# Autodesk Inventor assembly: 8 Omni Wheel
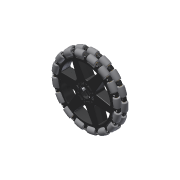
[picture p0: Inventor's stored thumbnail of the model, 180x180]
Saved by Autodesk Inventor 2013 (Build 170138000, 138)
## iProperties
Created: 2013-01-03
Part Number: 8 Omni Wheel
Document SubType Name: Assembly
Designer: Nemo
Author: Nemo
## Documents named in this file (6)
- H:\Nemo\Documents\Robotics\VexPro\Omni Wheel\8 Omni Wheel.iam
- H:\Nemo\Documents\Robotics\VexPro\Omni Wheel\Components\Omni Wheel Inside 8 in.ipt
- H:\Nemo\Documents\Robotics\VexPro\Omni Wheel\Components\Omni Wheel Outside 8 in.ipt
- H:\Nemo\Documents\Robotics\VexPro\Fasteners\Hex Standoff 8-32 x750.ipt
- H:\Nemo\Documents\Robotics\VexPro\Wheels\Components\Omni Roller 8 in.iam
- H:\Nemo\Documents\Robotics\VexPro\Omni Wheel\Components\Omni Wheel Screw for VexPro.ipt
## Components (73 placed, 5 different names)
1. Omni Wheel Inside 8 in:1 — Mate:1, Mate:3, Mate:4, Mate:5, Mate:7, Mate:8, Mate:10
2. Omni Wheel Outside 8 in:1 — Mate:1, Mate:3, Insert:1, Angle:1, Mate:6, Mate:11, Insert:2
3. Omni Wheel Outside 8 in:2 — Mate:4, Mate:5, Mate:6, Mate:7, Mate:9, Insert:3
4. Omni Roller 8 in:3 [sub-assembly] — Mate:10, Mate:11
5. Omni Roller 8 in:2 [sub-assembly] — Mate:8, Mate:9
6. Omni Wheel Screw for VexPro:1 — Insert:2
7. Omni Wheel Screw for VexPro:2 — Insert:3
8. Omni Roller 8 in:4 [sub-assembly]
9. Omni Roller 8 in:5 [sub-assembly]
10. Omni Wheel Screw for VexPro:3
11. Omni Wheel Screw for VexPro:18
12. Omni Roller 8 in:6 [sub-assembly]
13. Omni Roller 8 in:7 [sub-assembly]
14. Omni Wheel Screw for VexPro:4
15. Omni Wheel Screw for VexPro:19
16. Omni Roller 8 in:8 [sub-assembly]
17. Omni Roller 8 in:9 [sub-assembly]
18. Omni Wheel Screw for VexPro:5
19. Omni Wheel Screw for VexPro:20
20. Omni Roller 8 in:10 [sub-assembly]
21. Omni Roller 8 in:11 [sub-assembly]
22. Omni Wheel Screw for VexPro:6
23. Omni Wheel Screw for VexPro:21
24. Omni Roller 8 in:12 [sub-assembly]
25. Omni Roller 8 in:13 [sub-assembly]
26. Omni Wheel Screw for VexPro:7
27. Omni Wheel Screw for VexPro:22
28. Omni Roller 8 in:14 [sub-assembly]
29. Omni Roller 8 in:15 [sub-assembly]
30. Omni Wheel Screw for VexPro:8
31. Omni Wheel Screw for VexPro:23
32. Omni Roller 8 in:16 [sub-assembly]
33. Omni Roller 8 in:17 [sub-assembly]
34. Omni Wheel Screw for VexPro:9
35. Omni Wheel Screw for VexPro:24
36. Omni Roller 8 in:18 [sub-assembly]
37. Omni Roller 8 in:19 [sub-assembly]
38. Omni Wheel Screw for VexPro:10
39. Omni Wheel Screw for VexPro:25
40. Omni Roller 8 in:20 [sub-assembly]
41. Omni Roller 8 in:21 [sub-assembly]
42. Omni Wheel Screw for VexPro:11
43. Omni Wheel Screw for VexPro:26
44. Omni Roller 8 in:22 [sub-assembly]
45. Omni Roller 8 in:23 [sub-assembly]
46. Omni Wheel Screw for VexPro:12
47. Omni Wheel Screw for VexPro:27
48. Omni Roller 8 in:24 [sub-assembly]
49. Omni Roller 8 in:25 [sub-assembly]
50. Omni Wheel Screw for VexPro:13
51. Omni Wheel Screw for VexPro:28
52. Omni Roller 8 in:26 [sub-assembly]
53. Omni Roller 8 in:27 [sub-assembly]
54. Omni Wheel Screw for VexPro:14
55. Omni Wheel Screw for VexPro:29
56. Omni Roller 8 in:28 [sub-assembly]
57. Omni Roller 8 in:29 [sub-assembly]
58. Omni Wheel Screw for VexPro:15
59. Omni Wheel Screw for VexPro:30
60. Omni Roller 8 in:30 [sub-assembly]
61. Omni Roller 8 in:31 [sub-assembly]
62. Omni Wheel Screw for VexPro:16
63. Omni Wheel Screw for VexPro:31
64. Omni Roller 8 in:32 [sub-assembly]
65. Omni Roller 8 in:33 [sub-assembly]
66. Omni Wheel Screw for VexPro:17
67. Omni Wheel Screw for VexPro:32
68. Hex Standoff 8-32 x750:1 — Insert:1, Angle:1
69. Hex Standoff 8-32 x750:2
70. Hex Standoff 8-32 x750:3
71. Hex Standoff 8-32 x750:4
72. Hex Standoff 8-32 x750:5
73. Hex Standoff 8-32 x750:6
## Component patterns: (16 elements, first: Omni Roller 8 in:3 + Omni Roller 8 in:2 + Omni Wheel Screw for VexPro:1 + Omni Wheel Screw for VexPro:2), (6 elements, first: Hex Standoff 8-32 x750:1)
## Relationships (14: Mate 10, Insert 3, Angle 1)
- Mate:1: Omni Wheel Inside 8 in:1 ↔ Omni Wheel Outside 8 in:1
- Mate:3: Omni Wheel Inside 8 in:1 ↔ Omni Wheel Outside 8 in:1
- Insert:1: Omni Wheel Outside 8 in:1 ↔ Hex Standoff 8-32 x750:1
- Angle:1 (0 deg): Omni Wheel Outside 8 in:1 ↔ Hex Standoff 8-32 x750:1
- Mate:4: Omni Wheel Inside 8 in:1 ↔ Omni Wheel Outside 8 in:2
- Mate:5: Omni Wheel Inside 8 in:1 ↔ Omni Wheel Outside 8 in:2
- Mate:6: Omni Wheel Outside 8 in:1 ↔ Omni Wheel Outside 8 in:2
- Mate:7: Omni Wheel Inside 8 in:1 ↔ Omni Wheel Outside 8 in:2
- Mate:8: Omni Wheel Inside 8 in:1 ↔ Omni Roller 8 in:2
- Mate:9 (0.2286 mm): Omni Wheel Outside 8 in:2 ↔ Omni Roller 8 in:2
- Mate:10: Omni Wheel Inside 8 in:1 ↔ Omni Roller 8 in:3
- Mate:11 (0.2286 mm): Omni Wheel Outside 8 in:1 ↔ Omni Roller 8 in:3
- Insert:2: Omni Wheel Outside 8 in:1 ↔ Omni Wheel Screw for VexPro:1
- Insert:3: Omni Wheel Outside 8 in:2 ↔ Omni Wheel Screw for VexPro:2
